# Autodesk Inventor assembly: RpiTower
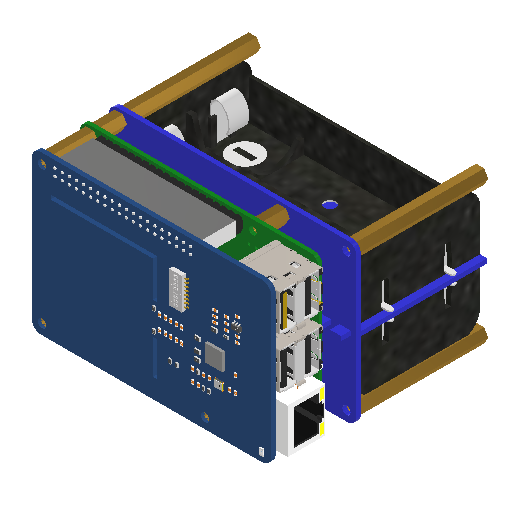
[picture p0: Inventor's stored thumbnail of the model, 512x512]
Saved by Autodesk Inventor 2025.2 (Build 292293000, 293)
## iProperties
Created: 2025-03-07
Part Number: RpiTower
Document SubType Name: Assembly
Designer: ahorat
Author: ahorat
## Documents named in this file (5)
- C:\Daten\Temp\R32EntrySystem\cad\RpiTower.iam
- C:\Daten\Temp\R32EntrySystem\cad\Rpi\Raspberry Pi 3.ipt
- C:\Daten\Temp\R32EntrySystem\cad\NFC_HAT\pn532_nfc_hat_asm.iam
- C:\Daten\Temp\R32EntrySystem\cad\UPS_HAT_E\Spacer_16mm.ipt
- C:\Daten\Temp\R32EntrySystem\cad\UPS_HAT_E\UPS_HAT_E.iam
## Components (6 placed, 4 different names)
1. Raspberry Pi 3:1 — Mate:1, Mate:2, Mate:3, Mate:4, Mate:5, Mate:6, Insert:2, Insert:3, Insert:4
2. pn532_nfc_hat_asm:1 [sub-assembly] — Mate:1, Mate:2, Mate:3
3. UPS_HAT_E:1 [sub-assembly] — Mate:4, Mate:5, Mate:6
4. Spacer_16mm:2 — Insert:2
5. Spacer_16mm:3 — Insert:3
6. Spacer_16mm:4 — Insert:4
## Relationships (9: Mate 6, Insert 3)
- Mate:1: Raspberry Pi 3:1 ↔ pn532_nfc_hat_asm:1
- Mate:2: Raspberry Pi 3:1 ↔ pn532_nfc_hat_asm:1
- Mate:3: Raspberry Pi 3:1 ↔ pn532_nfc_hat_asm:1
- Mate:4: Raspberry Pi 3:1 ↔ UPS_HAT_E:1
- Mate:5: Raspberry Pi 3:1 ↔ UPS_HAT_E:1
- Mate:6: Raspberry Pi 3:1 ↔ UPS_HAT_E:1
- Insert:2: Raspberry Pi 3:1 ↔ Spacer_16mm:2
- Insert:3: Raspberry Pi 3:1 ↔ Spacer_16mm:3
- Insert:4: Raspberry Pi 3:1 ↔ Spacer_16mm:4
